# Autodesk Inventor assembly: EBF_900.1-top_w_cups
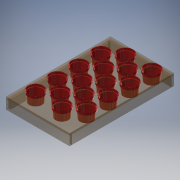
[picture p0: Inventor's stored thumbnail of the model, 180x180]
Saved by Autodesk Inventor 2019 (Build 230136000, 136)
## iProperties
Created: 2019-02-28
Part Number: EBF_900.1-top_w_cups
Document SubType Name: Assembly
Designer: Rene
Author: Rene
## Documents named in this file (6)
- C:\dev\c-scape\hardponics\dwg\eb_flow\EBF_900.1-top_w_cups.iam
- C:\dev\c-scape\hardponics\dwg\eb_flow\EBF_001.1-top-plate_cup-holder.ipt
- C:\dev\c-scape\hardponics\dwg\eb_flow\XGEN_sambal-bakje.ipt
- C:\dev\c-scape\hardponics\dwg\eb_flow\EBF_002.1-side-plate_cup-holder.ipt
- C:\dev\c-scape\hardponics\dwg\eb_flow\EBF_003.1-front-plate_cup-holder.ipt
- C:\dev\c-scape\hardponics\dwg\eb_flow\EBF_004.1-back-plate_cup-holder.ipt
## Components (21 placed, 5 different names)
1. EBF_001.1-top-plate_cup-holder:1 — Mate:1, Mate:2, Mate:3, Mate:4, Mate:5, Flush:1, Mate:6, Flush:2, Mate:7, Flush:3, Flush:4, Mate:10, Flush:5, Flush:6
2. EBF_002.1-side-plate_cup-holder:1 — Mate:5, Flush:1, Mate:8
3. EBF_002.1-side-plate_cup-holder:2 — Mate:6, Flush:2, Mate:9
4. EBF_003.1-front-plate_cup-holder:1 — Mate:7, Flush:3, Flush:4, Mate:8, Mate:9
5. EBF_004.1-back-plate_cup-holder:1 — Mate:10, Flush:5, Flush:6
6. XGEN_sambal-bakje:1 — Mate:1, Mate:2
7. XGEN_sambal-bakje:2 — Mate:3, Mate:4
8. XGEN_sambal-bakje:3
9. XGEN_sambal-bakje:4
10. XGEN_sambal-bakje:5
11. XGEN_sambal-bakje:6
12. XGEN_sambal-bakje:7
13. XGEN_sambal-bakje:8
14. XGEN_sambal-bakje:9
15. XGEN_sambal-bakje:10
16. XGEN_sambal-bakje:11
17. XGEN_sambal-bakje:12
18. XGEN_sambal-bakje:13
19. XGEN_sambal-bakje:14
20. XGEN_sambal-bakje:15
21. XGEN_sambal-bakje:16
## Component patterns: (8 elements, first: XGEN_sambal-bakje:1 + XGEN_sambal-bakje:2)
## Relationships (16: Mate 10, Flush 6)
- Mate:1: EBF_001.1-top-plate_cup-holder:1 ↔ XGEN_sambal-bakje:1
- Mate:2: EBF_001.1-top-plate_cup-holder:1 ↔ XGEN_sambal-bakje:1
- Mate:3: EBF_001.1-top-plate_cup-holder:1 ↔ XGEN_sambal-bakje:2
- Mate:4: EBF_001.1-top-plate_cup-holder:1 ↔ XGEN_sambal-bakje:2
- Mate:5: EBF_001.1-top-plate_cup-holder:1 ↔ EBF_002.1-side-plate_cup-holder:1
- Flush:1: EBF_001.1-top-plate_cup-holder:1 ↔ EBF_002.1-side-plate_cup-holder:1
- Mate:6: EBF_001.1-top-plate_cup-holder:1 ↔ EBF_002.1-side-plate_cup-holder:2
- Flush:2: EBF_001.1-top-plate_cup-holder:1 ↔ EBF_002.1-side-plate_cup-holder:2
- Mate:7: EBF_001.1-top-plate_cup-holder:1 ↔ EBF_003.1-front-plate_cup-holder:1
- Flush:3: EBF_001.1-top-plate_cup-holder:1 ↔ EBF_003.1-front-plate_cup-holder:1
- Flush:4: EBF_001.1-top-plate_cup-holder:1 ↔ EBF_003.1-front-plate_cup-holder:1
- Mate:8: EBF_002.1-side-plate_cup-holder:1 ↔ EBF_003.1-front-plate_cup-holder:1
- Mate:9: EBF_002.1-side-plate_cup-holder:2 ↔ EBF_003.1-front-plate_cup-holder:1
- Mate:10: EBF_001.1-top-plate_cup-holder:1 ↔ EBF_004.1-back-plate_cup-holder:1
- Flush:5: EBF_001.1-top-plate_cup-holder:1 ↔ EBF_004.1-back-plate_cup-holder:1
- Flush:6: EBF_001.1-top-plate_cup-holder:1 ↔ EBF_004.1-back-plate_cup-holder:1
